# Autodesk Inventor assembly: Turret Shooter Assembly
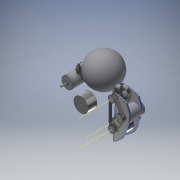
[picture p0: Inventor's stored thumbnail of the model, 180x180]
Saved by Autodesk Inventor 2019.4 (Build 234330000, 330)
## iProperties
Created: 2020-01-06
Part Number: Turret Shooter Assembly
Document SubType Name: Assembly
Designer: admin
Author: admin
## Documents named in this file (9)
- C:\Users\admin\Desktop\FRC 2020 Engineering\GitHub\7738-2020\Turret\Turret Shooter Assembly.iam
- C:\Users\admin\Desktop\FRC 2020 Engineering\GitHub\7738-2020\Turret\Omni Wheel\3_25_Omni-Directional_Wheel_217-4775.iam
- C:\Users\admin\Desktop\FRC 2020 Engineering\GitHub\7738-2020\Power Cell.ipt
- C:\Users\admin\Desktop\FRC 2020 Engineering\GitHub\7738-2020\Turret\Flywheel.ipt
- C:\Users\admin\Desktop\FRC 2020 Engineering\GitHub\7738-2020\Turret\Mini CIM\Mini_CIM_Motor_217-3371.ipt
- C:\Users\admin\Desktop\FRC 2020 Engineering\GitHub\7738-2020\CAD\Gearbox\F6800.ipt
- C:\Users\admin\Desktop\FRC 2020 Engineering\GitHub\7738-2020\Turret\Flywheel Bracket 1.ipt
- C:\Users\admin\Desktop\FRC 2020 Engineering\GitHub\7738-2020\Turret\Turret Shooter Assembly\Design Accelerator\Synchronous Belts Transmission3.iam
- C:\Users\admin\Desktop\FRC 2020 Engineering\GitHub\7738-2020\Turret\Flywheel Bracket 2.ipt
## Components (14 placed, 8 different names)
1. 3_25_Omni-Directional_Wheel_217-4775:1 [sub-assembly] — Flush:1, Angle:1, Mate:17, Flush:7
2. 3_25_Omni-Directional_Wheel_217-4775:2 [sub-assembly] — Flush:1, Mate:14
3. Power Cell:1 — Mate:5, Mate:6
4. Flywheel:1 — Flush:2, Mate:1, Flush:3, Mate:3, Flush:6, Mate:8, Flush:7, Mate:20, Mate:24
5. Flywheel:2 — Flush:2, Mate:1, Mate:4, Flush:4
6. Mini_CIM_Motor_217-3371:1 — Flush:3, Mate:9, Mate:10, Mate:18, Mate:21
7. Mini_CIM_Motor_217-3371:2 — Flush:4
8. F6800:2 — Mate:11, Mate:12
9. Flywheel Bracket 1:1 — Mate:8, Mate:9, Mate:10, Mate:11, Mate:12, Mate:25, Mate:27
10. Synchronous Belts Transmission:1 [sub-assembly] — Mate:18, Mate:19
11. Flywheel Bracket 2:1 — Mate:20, Mate:21, Mate:22, Mate:23, Mate:26, Mate:28
12. F6800:3 — Mate:22, Mate:23, Mate:24
13. F6800:4 — Mate:26, Mate:28
14. F6800:5 — Mate:25, Mate:27
## Relationships (31: Mate 23, Flush 7, Angle 1)
- Flush:1: 3_25_Omni-Directional_Wheel_217-4775:1 ↔ 3_25_Omni-Directional_Wheel_217-4775:2
- Flush:2: Flywheel:1 ↔ Flywheel:2
- Mate:1 (207 mm): Flywheel:1 ↔ Flywheel:2
- Flush:3 (-5 mm): Flywheel:1 ↔ Mini_CIM_Motor_217-3371:1
- Mate:3 (103.5 mm): Flywheel:1
- Mate:4 (-103.5 mm): Flywheel:2
- Mate:5: Power Cell:1
- Mate:6: Power Cell:1
- Flush:4 (-5 mm): Flywheel:2 ↔ Mini_CIM_Motor_217-3371:2
- Flush:5 (103.5 mm)
- Flush:6 (-25 mm): Flywheel:1
- Mate:8: Flywheel:1 ↔ Flywheel Bracket 1:1
- Mate:9: Mini_CIM_Motor_217-3371:1 ↔ Flywheel Bracket 1:1
- Mate:10: Mini_CIM_Motor_217-3371:1 ↔ Flywheel Bracket 1:1
- Mate:11: F6800:2 ↔ Flywheel Bracket 1:1
- Mate:12 (0.2 mm): F6800:2 ↔ Flywheel Bracket 1:1
- Angle:1 (0 deg): 3_25_Omni-Directional_Wheel_217-4775:1
- Mate:14 (-104.775 mm): 3_25_Omni-Directional_Wheel_217-4775:2
- Mate:17: 3_25_Omni-Directional_Wheel_217-4775:1
- Mate:18: Mini_CIM_Motor_217-3371:1 ↔ Synchronous Belts Transmission:1
- Mate:19: Synchronous Belts Transmission:1
- Flush:7 (5.95 mm): 3_25_Omni-Directional_Wheel_217-4775:1 ↔ Flywheel:1
- Mate:20: Flywheel:1 ↔ Flywheel Bracket 2:1
- Mate:21: Mini_CIM_Motor_217-3371:1 ↔ Flywheel Bracket 2:1
- Mate:22: Flywheel Bracket 2:1 ↔ F6800:3
- Mate:23 (0.2 mm): Flywheel Bracket 2:1 ↔ F6800:3
- Mate:24 (5 mm): Flywheel:1 ↔ F6800:3
- Mate:25: Flywheel Bracket 1:1 ↔ F6800:5
- Mate:26: Flywheel Bracket 2:1 ↔ F6800:4
- Mate:27 (0.2 mm): Flywheel Bracket 1:1 ↔ F6800:5
- Mate:28 (0.2 mm): Flywheel Bracket 2:1 ↔ F6800:4
